# Autodesk Inventor assembly: złożenie2
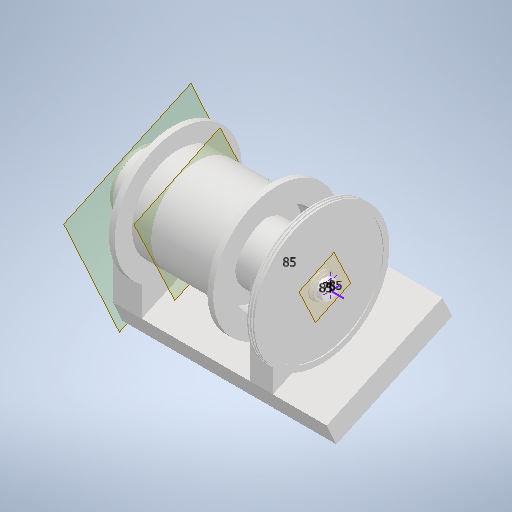
[picture p0: Inventor's stored thumbnail of the model, 512x512]
Saved by Autodesk Inventor 2025.2 (Build 292293000, 293)
## iProperties
Created: 2025-05-18
Part Number: złożenie2
Document SubType Name: Assembly
Designer: PC
Author: PC
## Documents named in this file (12)
- D:\Podstawy-Konstrukcji-Maszyn\Projekt3_temat3\src\Assemblies\złożenie2.iam
- D:\Podstawy-Konstrukcji-Maszyn\Projekt3_temat3\src\Parts\Wał4.ipt
- D:\Podstawy-Konstrukcji-Maszyn\Projekt3_temat3\src\Parts\1415151513515.ipt
- D:\Podstawy-Konstrukcji-Maszyn\Projekt3_temat3\src\ContentCenter\pl-PL\BS 290 SKF(05)\BS 290 SKF - SKF QJ 230 N2.ipt
- D:\Podstawy-Konstrukcji-Maszyn\Projekt3_temat3\src\Assemblies\Połączenie wpustowe1.iam
- D:\Podstawy-Konstrukcji-Maszyn\Projekt3_temat3\src\Assemblies\Połączenie wpustowe2.iam
- D:\Podstawy-Konstrukcji-Maszyn\Projekt3_temat3\src\Parts\podstawa.ipt
- D:\Podstawy-Konstrukcji-Maszyn\Projekt3_temat3\src\ContentCenter\pl-PL\DIN 705   B\DIN 705 - B150.ipt
- D:\Podstawy-Konstrukcji-Maszyn\Projekt3_temat3\src\Parts\pięćśetka.ipt
- D:\Podstawy-Konstrukcji-Maszyn\Projekt3_temat3\src\ContentCenter\pl-PL\AS 1110\AS 1110 - M36 x 60.ipt
- D:\Podstawy-Konstrukcji-Maszyn\Projekt3_temat3\src\ContentCenter\pl-PL\DIN 3760 A\DIN 3760 - A - 150 x 180 x 15 - NBR.ipt
- D:\Podstawy-Konstrukcji-Maszyn\Projekt3_temat3\src\Parts\koło zębate2 (1).ipt
## Components (22 placed, 10 different names)
1. Wał:1 — Równoległe:1, Zestawiające:4, Kątowe:3, Kątowe:5, Kątowe:9, Równoległe:7, Równoległe:9, Kątowe:11, Zestawiające:11, Równoległe:10, Kątowe:12, Zestawiające:12, Równoległe:11, Kątowe:13, Zestawiające:13
2. 1415151513515:1 — Zestawiające:4, Kątowe:3, Kątowe:5, Kątowe:9
3. BS 290 SKF- do styku czteropunktowego SKF QJ 230 N2:1 — Obrotowe:1
4. BS 290 SKF- do styku czteropunktowego SKF QJ 230 N2:2 — Walcowe:1, Obrotowe:2
5. Połączenie wpustowe:1 [sub-assembly] — Równoległe:9, Kątowe:11, Zestawiające:11
6. Połączenie wpustowe:2 [sub-assembly] — Równoległe:10, Kątowe:12, Zestawiające:12
7. podstawa:1 — Walcowe:1, Obrotowe:3, Obrotowe:4, Obrotowe:5, Obrotowe:6, Obrotowe:7, Obrotowe:8, Obrotowe:9, Obrotowe:10, Obrotowe:12
8. DIN 705 B B150:1 — Obrotowe:1
9. DIN 705 B B150:2 — Obrotowe:2
10. pięćśetka:1 — Obrotowe:3
11. AS 1110 - Metryczny M36 x 60:1 — Obrotowe:7
12. AS 1110 - Metryczny M36 x 60:2 — Obrotowe:5
13. AS 1110 - Metryczny M36 x 60:3 — Obrotowe:6
14. AS 1110 - Metryczny M36 x 60:4 — Obrotowe:4
15. DIN 3760 A A - 150 x 180 x 15 - NBR:1
16. pięćśetka:2 — Obrotowe:8, Obrotowe:11
17. AS 1110 - Metryczny M36 x 60:5 — Obrotowe:10
18. AS 1110 - Metryczny M36 x 60:6 — Obrotowe:9
19. AS 1110 - Metryczny M36 x 60:7 — Obrotowe:11
20. AS 1110 - Metryczny M36 x 60:8 — Obrotowe:12
21. koło zębate2 (1):1
22. Połączenie wpustowe:3 [sub-assembly] — Równoległe:11, Kątowe:13, Zestawiające:13
## Relationships (29: RevoluteJoint 12, Flush 6, Angle 6, Mate 4, CylindricalJoint 1)
- Równoległe:1 [Flush]: Wał:1
- Równoległe:2 [Flush] (-200 mm)
- Zestawiające:4 [Mate] (180 mm): Wał:1 ↔ 1415151513515:1
- Kątowe:3 [Angle] (90 deg): Wał:1 ↔ 1415151513515:1
- Kątowe:5 [Angle] (90 deg): Wał:1 ↔ 1415151513515:1
- Kątowe:9 [Angle] (90 deg): Wał:1 ↔ 1415151513515:1
- Walcowe:1 [CylindricalJoint]: BS 290 SKF- do styku czteropunktowego SKF QJ 230 N2:2 ↔ podstawa:1
- Obrotowe:1 [RevoluteJoint]: BS 290 SKF- do styku czteropunktowego SKF QJ 230 N2:1 ↔ DIN 705 B B150:1
- Obrotowe:2 [RevoluteJoint]: BS 290 SKF- do styku czteropunktowego SKF QJ 230 N2:2 ↔ DIN 705 B B150:2
- Obrotowe:3 [RevoluteJoint]: podstawa:1 ↔ pięćśetka:1
- Obrotowe:4 [RevoluteJoint]: podstawa:1 ↔ AS 1110 - Metryczny M36 x 60:4
- Obrotowe:5 [RevoluteJoint]: podstawa:1 ↔ AS 1110 - Metryczny M36 x 60:2
- Obrotowe:6 [RevoluteJoint]: podstawa:1 ↔ AS 1110 - Metryczny M36 x 60:3
- Obrotowe:7 [RevoluteJoint]: podstawa:1 ↔ AS 1110 - Metryczny M36 x 60:1
- Obrotowe:8 [RevoluteJoint]: podstawa:1 ↔ pięćśetka:2
- Obrotowe:9 [RevoluteJoint] (-35 mm): podstawa:1 ↔ AS 1110 - Metryczny M36 x 60:6
- Obrotowe:10 [RevoluteJoint] (35 mm): podstawa:1 ↔ AS 1110 - Metryczny M36 x 60:5
- Obrotowe:11 [RevoluteJoint] (-35 mm): pięćśetka:2 ↔ AS 1110 - Metryczny M36 x 60:7
- Obrotowe:12 [RevoluteJoint]: podstawa:1 ↔ AS 1110 - Metryczny M36 x 60:8
- Równoległe:7 [Flush] (-50 mm): Wał:1
- Równoległe:9 [Flush] (204.9231 mm): Wał:1 ↔ Połączenie wpustowe:1
- Kątowe:11 [Angle] (180 deg): Wał:1 ↔ Połączenie wpustowe:1
- Zestawiające:11 [Mate]: Wał:1 ↔ Połączenie wpustowe:1
- Równoległe:10 [Flush] (204.9722 mm): Wał:1 ↔ Połączenie wpustowe:2
- Kątowe:12 [Angle] (0 deg): Wał:1 ↔ Połączenie wpustowe:2
- Zestawiające:12 [Mate]: Wał:1 ↔ Połączenie wpustowe:2
- Równoległe:11 [Flush] (56.6721 mm): Wał:1 ↔ Połączenie wpustowe:3
- Kątowe:13 [Angle] (180 deg): Wał:1 ↔ Połączenie wpustowe:3
- Zestawiające:13 [Mate]: Wał:1 ↔ Połączenie wpustowe:3
